# Autodesk Inventor assembly: Plate2.0Assembly
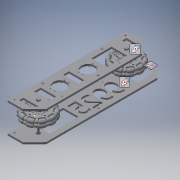
[picture p0: Inventor's stored thumbnail of the model, 180x180]
Saved by Autodesk Inventor 2017 (Build 210142000, 142)
## iProperties
Created: 2017-08-08
Part Number: Plate2.0Assembly
Document SubType Name: Assembly
Designer: User
Author: User
## Documents named in this file (4)
- C:\Robotics\CAD\2016-17_CAD\Plate2.0Assembly.iam
- C:\Robotics\CAD\2016-17_CAD\DriveTrain\DrainTrainPlate2.0LeftOutside.iam
- C:\Robotics\CAD\2016-17_CAD\DriveTrain\DriveTrainPlate2.0LeftInside.ipt
- C:\Robotics\CAD\2016-17_CAD\DriveTrain\wheel sub assemblly omni wheels.iam
## Components (4 placed, 3 different names)
1. DrainTrainPlate2.0LeftOutside:1 [sub-assembly] — Mate:5, Mate:6
2. DriveTrainPlate2.0LeftInside:1 — Mate:1, Mate:2, Mate:3, Mate:4
3. wheel sub assemblly omni wheels:1 [sub-assembly] — Mate:1, Mate:2, Mate:6
4. wheel sub assemblly omni wheels:2 [sub-assembly] — Mate:3, Mate:4, Mate:5
## Relationships (6: Mate 6)
- Mate:1: DriveTrainPlate2.0LeftInside:1 ↔ wheel sub assemblly omni wheels:1
- Mate:2: DriveTrainPlate2.0LeftInside:1 ↔ wheel sub assemblly omni wheels:1
- Mate:3: DriveTrainPlate2.0LeftInside:1 ↔ wheel sub assemblly omni wheels:2
- Mate:4: DriveTrainPlate2.0LeftInside:1 ↔ wheel sub assemblly omni wheels:2
- Mate:5: DrainTrainPlate2.0LeftOutside:1 ↔ wheel sub assemblly omni wheels:2
- Mate:6: DrainTrainPlate2.0LeftOutside:1 ↔ wheel sub assemblly omni wheels:1
